# Autodesk Inventor assembly: DelrinY-Wheel-Bottom_MIR
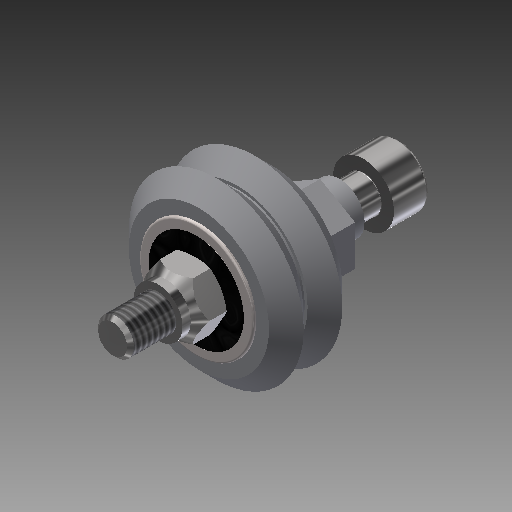
[picture p0: Inventor's stored thumbnail of the model, 512x512]
Saved by Autodesk Inventor 2017 (Build 210142000, 142)
## iProperties
Created: 2016-07-20
Part Number: DelrinY-Wheel-Bottom_MIR
Document SubType Name: Assembly
Designer: User
Author: User
## Documents named in this file (5)
- C:\All INVENTOR\SL-Inventor\SL-Beast 3D Printer\DelrinY-Wheel-Bottom_MIR.iam
- C:\All INVENTOR\SL-Inventor\SL-Beast 3D Printer\DelrinWheel_MIR.iam
- C:\All INVENTOR\SL-Inventor\SL-Beast 3D Printer\en-US\ANSI B18.3.1M(6)\ANSI B18.3.1M - M5x0.8 x 35(1).ipt
- C:\All INVENTOR\SL-Inventor\SL-Beast 3D Printer\en-US\ANSI B18.16.3M(2)\ANSI B18.16.3M - Property Class 5 and 10 - Metric M5 x 0.8 Metal Type.ipt
- C:\All INVENTOR\SL-Inventor\SL-Beast 3D Printer\Eccentric Spacer_MIR.ipt
## Components (4 placed, 4 different names)
1. DelrinWheel_MIR:1 [sub-assembly] — Insert:1, Flush:1
2. Forged Socket Head Cap Screw - Metric M5x0.8 x 35:1
3. Prevailing Torque Type Hex Nut - Steel Metric Property Class 5 and 10 - Metric M5 x 0.8 Metal Type:1 — Insert:1
4. Eccentric Spacer_MIR:1 — Flush:1
## Relationships (2: Insert 1, Mate 1)
- Insert:1: DelrinWheel_MIR:1 ↔ Prevailing Torque Type Hex Nut - Steel Metric Property Class 5 and 10 - Metric M5 x 0.8 Metal Type:1
- Flush:1 [Mate]: DelrinWheel_MIR:1 ↔ Eccentric Spacer_MIR:1
